# Autodesk Inventor assembly: intake
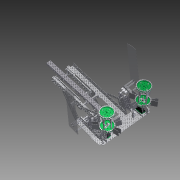
[picture p0: Inventor's stored thumbnail of the model, 180x180]
Saved by Autodesk Inventor 2014 SP1 (Build 180222100, 222)
## iProperties
Created: 2014-04-04
Part Number: intake
Document SubType Name: Assembly
Designer: Ryan
Author: Ryan
## Documents named in this file (5)
- C:\Users\Ryan\Desktop\sw\toss up 5th A bot\intake\intake.iam
- C:\Users\Ryan\Desktop\sw\toss up 5th A bot\intake\flip down asmb.iam
- C:\Users\Ryan\Desktop\sw\toss up 5th A bot\intake\6 bar attachment.iam
- C:\Users\Ryan\Desktop\sw\toss up 5th A bot\intake\sled.iam
- C:\Users\Ryan\Desktop\sw\toss up 5th A bot\intake\6 bar attachment_MIR.iam
## Components (4 placed, 4 different names)
1. flip down asmb:1 [sub-assembly] — Mate:5, Mate:6
2. 6 bar attachment:1 [sub-assembly] — Mate:1, Mate:2, Mate:3, Mate:4, Mate:5, Mate:6, Mate:7, Mate:8
3. sled:1 [sub-assembly] — Mate:1, Mate:2, Mate:3, Mate:4, Mate:9
4. 6 bar attachment_MIR:1 [sub-assembly] — Mate:7, Mate:8, Mate:9
## Relationships (9: Mate 9)
- Mate:1 (2.3114 mm): 6 bar attachment:1 ↔ sled:1
- Mate:2 (2.3114 mm): 6 bar attachment:1 ↔ sled:1
- Mate:3: 6 bar attachment:1 ↔ sled:1
- Mate:4 (10.8458 mm): 6 bar attachment:1 ↔ sled:1
- Mate:5: flip down asmb:1 ↔ 6 bar attachment:1
- Mate:6: flip down asmb:1 ↔ 6 bar attachment:1
- Mate:7: 6 bar attachment:1 ↔ 6 bar attachment_MIR:1
- Mate:8: 6 bar attachment:1 ↔ 6 bar attachment_MIR:1
- Mate:9: sled:1 ↔ 6 bar attachment_MIR:1
## Named parameters: q = 2.3114 mm
